# Autodesk Inventor assembly: 자동 커튼
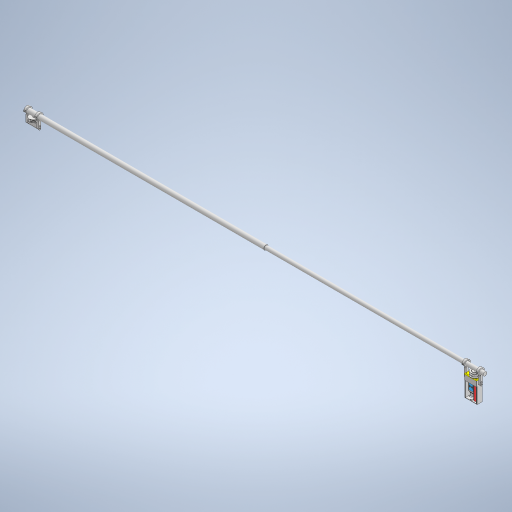
[picture p0: Inventor's stored thumbnail of the model, 512x512]
Saved by Autodesk Inventor 2023.1 (Build 271208000, 208)
## iProperties
Created: 2022-09-03
Part Number: 자동 커튼
Document SubType Name: Assembly
Designer: fly01
Author: fly01
## Documents named in this file (16)
- C:\Users\fly01\Desktop\IOT부품\커튼\자동 커튼.iam
- C:\Users\fly01\Desktop\IOT부품\커튼\감속기어 모터'.ipt
- C:\Users\fly01\Desktop\IOT부품\커튼\모터 드라이버.ipt
- C:\Users\fly01\Desktop\IOT부품\커튼\커튼 서보 커버.ipt
- C:\Users\fly01\Desktop\IOT부품\커튼\커튼 정면 커버.ipt
- C:\Users\fly01\Desktop\IOT부품\커튼\커튼 하우징.ipt
- C:\Users\fly01\Desktop\IOT부품\커튼\커튼 휠.ipt
- C:\Users\fly01\Desktop\IOT부품\18650배터리.ipt
- C:\Users\fly01\Desktop\IOT부품\esp32f.ipt
- C:\Users\fly01\Desktop\IOT부품\커튼\커튼 봉.ipt
- C:\Users\fly01\Desktop\IOT부품\커튼\봉걸이.ipt
- C:\Users\fly01\Desktop\IOT부품\커튼\봉걸이 반대편.ipt
- C:\Users\fly01\Desktop\IOT부품\커튼\회전 축 고정대 봉걸이1.ipt
- C:\Users\fly01\Desktop\IOT부품\커튼\회전 축 고정대 봉걸이2.ipt
- C:\Users\fly01\Desktop\IOT부품\커튼\회전 축 고정대.ipt
- C:\Users\fly01\Desktop\IOT부품\커튼\회전 축 휠.ipt
## Components (15 placed, 15 different names)
1. 감속기어 모터':1 — 삽입:1, 삽입:2, 삽입:8
2. 모터 드라이버:1 — 메이트:4
3. 커튼 서보 커버:1 — 삽입:3, 삽입:4
4. 커튼 정면 커버:1 — 메이트:2, 메이트:3, 메이트:5, 각도:2
5. 커튼 하우징:1 — 메이트:1, 메이트:2, 메이트:3, 삽입:1, 삽입:2, 삽입:3, 삽입:4, 삽입:5, 삽입:6, 삽입:7, 메이트:5, 각도:1, 삽입:9, 삽입:11, 삽입:15
6. 커튼 휠:1 — 삽입:8
7. 18650배터리:1 — 삽입:5
8. esp32f:1 — 삽입:6, 삽입:7, 메이트:4
9. 커튼 봉:1 — 각도:1, 삽입:10, 삽입:14
10. 봉걸이:1 — 삽입:9, 삽입:10, 삽입:15
11. 봉걸이 반대편:1 — 삽입:11
12. 회전 축 고정대 봉걸이1:1 — 삽입:14, 삽입:16, 삽입:17
13. 회전 축 고정대 봉걸이2:1 — 삽입:19
14. 회전 축 고정대:1 — 삽입:16, 삽입:17, 삽입:19, 각도:2, 삽입:20
15. 회전 축 휠:1 — 삽입:20
## Relationships (24: Insert 17, Mate 5, Angle 2)
- 메이트:1 [Mate]: 커튼 하우징:1
- 메이트:2 [Mate]: 커튼 정면 커버:1 ↔ 커튼 하우징:1
- 메이트:3 [Mate]: 커튼 정면 커버:1 ↔ 커튼 하우징:1
- 삽입:1 [Insert]: 감속기어 모터':1 ↔ 커튼 하우징:1
- 삽입:2 [Insert]: 감속기어 모터':1 ↔ 커튼 하우징:1
- 삽입:3 [Insert]: 커튼 서보 커버:1 ↔ 커튼 하우징:1
- 삽입:4 [Insert]: 커튼 서보 커버:1 ↔ 커튼 하우징:1
- 삽입:5 [Insert] (3 mm): 커튼 하우징:1 ↔ 18650배터리:1
- 삽입:6 [Insert]: 커튼 하우징:1 ↔ esp32f:1
- 삽입:7 [Insert]: 커튼 하우징:1 ↔ esp32f:1
- 메이트:4 [Mate]: 모터 드라이버:1 ↔ esp32f:1
- 메이트:5 [Mate]: 커튼 정면 커버:1 ↔ 커튼 하우징:1
- 삽입:8 [Insert]: 감속기어 모터':1 ↔ 커튼 휠:1
- 각도:1 [Angle] (0 deg): 커튼 하우징:1 ↔ 커튼 봉:1
- 삽입:9 [Insert]: 커튼 하우징:1 ↔ 봉걸이:1
- 삽입:10 [Insert] (-100 mm): 커튼 봉:1 ↔ 봉걸이:1
- 삽입:11 [Insert]: 커튼 하우징:1 ↔ 봉걸이 반대편:1
- 삽입:14 [Insert]: 커튼 봉:1 ↔ 회전 축 고정대 봉걸이1:1
- 삽입:15 [Insert]: 커튼 하우징:1 ↔ 봉걸이:1
- 삽입:16 [Insert]: 회전 축 고정대 봉걸이1:1 ↔ 회전 축 고정대:1
- 삽입:17 [Insert]: 회전 축 고정대 봉걸이1:1 ↔ 회전 축 고정대:1
- 삽입:19 [Insert]: 회전 축 고정대 봉걸이2:1 ↔ 회전 축 고정대:1
- 각도:2 [Angle] (0 deg): 커튼 정면 커버:1 ↔ 회전 축 고정대:1
- 삽입:20 [Insert] (0.25 mm): 회전 축 고정대:1 ↔ 회전 축 휠:1
